# Autodesk Inventor assembly: PiWithCase-SubAssembly
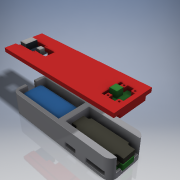
[picture p0: Inventor's stored thumbnail of the model, 180x180]
Saved by Autodesk Inventor 2019 (Build 230136000, 136)
## iProperties
Created: 2019-04-12
Part Number: PiWithCase-SubAssembly
Document SubType Name: Assembly
Designer: Epsilon
Author: Epsilon
## Documents named in this file (9)
- F:\Code\3D-Scanner-Hardware\Assembly\PiWithCase-SubAssembly.iam
- F:\Code\3D-Scanner-Hardware\PiHolder.ipt
- F:\Code\3D-Scanner-Hardware\ExistingParts\RaspberryPi0W-SafeSpecs.ipt
- F:\Code\3D-Scanner-Hardware\ExistingParts\4400mAh-LiIon-Battery.ipt
- F:\Code\3D-Scanner-Hardware\ExistingParts\Adafruit-PowerBoost500.ipt
- F:\Code\3D-Scanner-Hardware\ExistingParts\RaspberryPi0W-BerryIMUV3-SafeSpecs.ipt
- F:\Code\3D-Scanner-Hardware\ExistingParts\RaspberryPiCamera.ipt
- F:\Code\3D-Scanner-Hardware\ExistingParts\Adafruit-MicroLipoBatteryCharger.ipt
- F:\Code\3D-Scanner-Hardware\Cap.ipt
## Components (8 placed, 8 different names)
1. PiHolder:1 — Mate:1, Mate:2, Mate:3, Mate:4, Mate:5, Tangent:1, Mate:12, Mate:13, Mate:14
2. RaspberryPi0W-SafeSpecs:1 — Mate:1, Mate:2, Mate:3, Mate:9, Mate:10, Mate:11
3. 4400mAh-LiIon-Battery:1 — Mate:4, Mate:5, Tangent:1
4. Adafruit-PowerBoost500:1 — Mate:18, Mate:19, Mate:20
5. RaspberryPi0W-BerryIMUV3-SafeSpecs:1 — Mate:9, Mate:10, Mate:11
6. RaspberryPiCamera:1 — Mate:15, Mate:16, Mate:17
7. Adafruit-MicroLipoBatteryCharger:1
8. Cap:1 — Mate:12, Mate:13, Mate:14, Mate:15, Mate:16, Mate:17, Mate:18, Mate:19, Mate:20
## Relationships (18: Mate 17, Tangent 1)
- Mate:1: PiHolder:1 ↔ RaspberryPi0W-SafeSpecs:1
- Mate:2: PiHolder:1 ↔ RaspberryPi0W-SafeSpecs:1
- Mate:3: PiHolder:1 ↔ RaspberryPi0W-SafeSpecs:1
- Mate:4: PiHolder:1 ↔ 4400mAh-LiIon-Battery:1
- Mate:5: PiHolder:1 ↔ 4400mAh-LiIon-Battery:1
- Tangent:1: PiHolder:1 ↔ 4400mAh-LiIon-Battery:1
- Mate:9: RaspberryPi0W-SafeSpecs:1 ↔ RaspberryPi0W-BerryIMUV3-SafeSpecs:1
- Mate:10: RaspberryPi0W-SafeSpecs:1 ↔ RaspberryPi0W-BerryIMUV3-SafeSpecs:1
- Mate:11: RaspberryPi0W-SafeSpecs:1 ↔ RaspberryPi0W-BerryIMUV3-SafeSpecs:1
- Mate:12 (50.8 mm): PiHolder:1 ↔ Cap:1
- Mate:13: PiHolder:1 ↔ Cap:1
- Mate:14: PiHolder:1 ↔ Cap:1
- Mate:15: RaspberryPiCamera:1 ↔ Cap:1
- Mate:16: RaspberryPiCamera:1 ↔ Cap:1
- Mate:17: RaspberryPiCamera:1 ↔ Cap:1
- Mate:18: Adafruit-PowerBoost500:1 ↔ Cap:1
- Mate:19: Adafruit-PowerBoost500:1 ↔ Cap:1
- Mate:20: Adafruit-PowerBoost500:1 ↔ Cap:1
